# Autodesk Inventor assembly: v1_assem
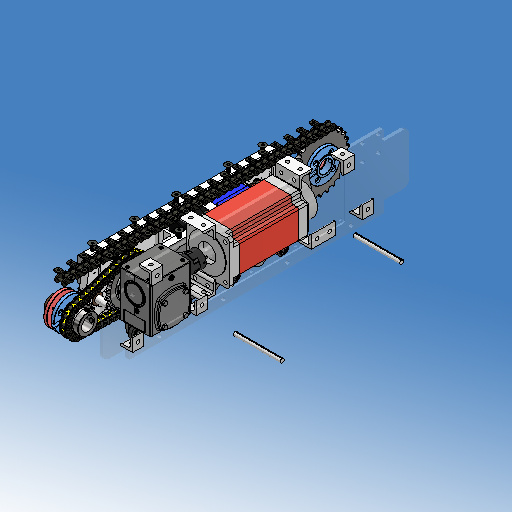
[picture p0: Inventor's stored thumbnail of the model, 512x512]
Saved by Autodesk Inventor 2025 (Build 290162000, 162)
## iProperties
Created: 2022-07-26
Part Number: v1_assem
Document SubType Name: Assembly
Designer: kumpu
Mass: 23927.4 g
Surface Area: 24107.2 cm^2
Volume: 6864.77 cm^3
Author: kumpu
## Documents named in this file (57)
- C:\Users\seene\OneDrive\SBRT\Robocup Rescue\Drive\v1\v1_assem.iam
- C:\Users\seene\OneDrive\SBRT\Robocup Rescue\Drive\v1\Placeholder_ChassisMain.ipt
- C:\Users\seene\OneDrive\SBRT\Robocup Rescue\Drive\v1\5887K172_Right-Angle Speed Reducer.ipt
- C:\Users\seene\OneDrive\SBRT\Robocup Rescue\Drive\v1\QCI-34HC-3_v2.ipt
- C:\Users\seene\OneDrive\SBRT\Robocup Rescue\Drive\v1\Dimensions(Roughly).ipt
- C:\Users\seene\OneDrive\SBRT\Robocup Rescue\Drive\v1\3 Stage HD - CIM Sport.iam
- C:\Users\seene\OneDrive\SBRT\Robocup Rescue\Drive\v1\50XX.ipt
- C:\Users\seene\OneDrive\SBRT\Robocup Rescue\Drive\v1\9939T12_Durometer 64D Spider for 1-5 16 OD Set Screw Vibrate-Damping Precision Flexible Shaft Coupling.ipt
- C:\Users\seene\OneDrive\SBRT\Robocup Rescue\Drive\v1\9939T102_Vibrate-Damping Precision Flexible Shaft Coupling.ipt
- C:\Users\seene\OneDrive\SBRT\Robocup Rescue\Drive\v1\9939T104_Vibrate-Damping Precision Flexible Shaft Coupling.ipt
- C:\Users\seene\OneDrive\SBRT\Robocup Rescue\Drive\v1\Bevels_assem.iam
- C:\Users\seene\OneDrive\SBRT\Robocup Rescue\Drive\v1\ChassisInterface.ipt
- C:\Users\seene\OneDrive\SBRT\Robocup Rescue\Drive\v1\TopPlate.ipt
- C:\Users\seene\OneDrive\SBRT\Robocup Rescue\Drive\v1\6836N166_Flat Sprocket.ipt
- C:\Users\seene\OneDrive\SBRT\Robocup Rescue\Drive\v1\2299K28_Flat Sprocket.ipt
- C:\Users\seene\OneDrive\SBRT\Robocup Rescue\Drive\v1\am-0077a 500 Key Hub REV3.ipt
- C:\Users\seene\OneDrive\SBRT\Robocup Rescue\Drive\v1\6280K675_Roller Chain Sprocket.ipt
- C:\Users\seene\OneDrive\SBRT\Robocup Rescue\Drive\v1\95412A316_18-8 Stainless Steel Threaded Rod.ipt
- C:\Users\seene\OneDrive\SBRT\Robocup Rescue\Drive\v1\91259A585_Alloy Steel Shoulder Screw.ipt
- C:\Users\seene\OneDrive\SBRT\Robocup Rescue\Drive\v1\96505A116_Steel Oversized Washer.ipt
- C:\Users\seene\OneDrive\SBRT\Robocup Rescue\Drive\v1\96282A101_High-Strength Steel Serrated Flange Locknut.ipt
- C:\Users\seene\OneDrive\SBRT\Robocup Rescue\Drive\v1\rubberWasher1.ipt
- C:\Users\seene\OneDrive\SBRT\Robocup Rescue\Drive\v1\trackpath.ipt
- C:\Users\seene\OneDrive\SBRT\Robocup Rescue\Drive\v1\Flipper\chain_male v7.ipt
- C:\Users\seene\OneDrive\SBRT\Robocup Rescue\Drive\v1\Flipper\chain_female v7.ipt
- C:\Users\seene\OneDrive\SBRT\Robocup Rescue\Drive\v1\5055MotorBlock.ipt
- C:\Users\seene\OneDrive\SBRT\Robocup Rescue\Drive\v1\7779T391_Low-Carbon Steel U-Channel.ipt
- C:\Users\seene\OneDrive\SBRT\Robocup Rescue\Drive\v1\am-2460 35 Tooth CIM Gear.ipt
- C:\Users\seene\OneDrive\SBRT\Robocup Rescue\Drive\v1\Flipper\rigid mount shoulder side.ipt
- C:\Users\seene\OneDrive\SBRT\Robocup Rescue\Drive\v1\Flipper\rigid mount threaded side.ipt
- C:\Users\seene\OneDrive\SBRT\Robocup Rescue\Drive\v1\57155K324_Stainless Steel Ball Bearing.ipt
- C:\Users\seene\OneDrive\SBRT\Robocup Rescue\Drive\v1\Spur Gear (28 teeth).ipt
- C:\Users\seene\OneDrive\SBRT\Robocup Rescue\Drive\v1\am-2352 50 Tooth 20 DP 0.75 in. Hex Bore Steel Gear.ipt
- C:\Users\seene\OneDrive\SBRT\Robocup Rescue\Drive\v1\V-Slot wheel.ipt
- C:\Users\seene\OneDrive\SBRT\Robocup Rescue\Drive\v1\91239A241_Button Head Hex Drive Screw.ipt
- C:\Users\seene\OneDrive\SBRT\Robocup Rescue\Drive\v1\6153K15_Stainless Steel Ball Bearing.ipt
- C:\Users\seene\OneDrive\SBRT\Robocup Rescue\Drive\v1\98688A115_General Purpose Zinc-Plated Steel Washer.ipt
- C:\Users\seene\OneDrive\SBRT\Robocup Rescue\Drive\v1\4416T771_Easy-to-Machine 1215 Carbon Steel.ipt
- C:\Users\seene\OneDrive\SBRT\Robocup Rescue\Drive\v1\2868T203_High-Load Oil-Embedded 863 Sleeve Bearing.ipt
- C:\Users\seene\OneDrive\SBRT\Robocup Rescue\Drive\v1\1439K211_1045 Carbon Steel Keyed Rotary Shaft.ipt
- C:\Users\seene\OneDrive\SBRT\Robocup Rescue\Drive\v1\am-0185 45 Tooth Gear 20 dp 500 Hex Bore.ipt
- C:\Users\seene\OneDrive\SBRT\Robocup Rescue\Drive\v1\2938T738_High-Load Oil-Embedded Sleeve Bearing.ipt
- C:\Users\seene\OneDrive\SBRT\Robocup Rescue\Drive\v1\2868T9_High-Load Oil-Embedded 863 Sleeve Bearing.ipt
- C:\Users\seene\OneDrive\SBRT\Robocup Rescue\Drive\v1\2938T12_High-Load Oil-Embedded Sleeve Bearing.ipt
- C:\Users\seene\OneDrive\SBRT\Robocup Rescue\Drive\v1\97175A383_Pull-Out Dowel Pin.ipt
- C:\Users\seene\OneDrive\SBRT\Robocup Rescue\Drive\v1\47065T236_Silver Corner Bracket.ipt
- C:\Users\seene\OneDrive\SBRT\Robocup Rescue\Drive\v1\47065T237_T-Slotted Framing.ipt
- C:\Users\seene\OneDrive\SBRT\Robocup Rescue\Drive\v1\40 chain link.ipt
- C:\Users\seene\OneDrive\SBRT\Robocup Rescue\Drive\v1\ChainPath.ipt
- C:\Users\seene\OneDrive\SBRT\Robocup Rescue\Drive\v1\OuterDriveRail.ipt
- C:\Users\seene\OneDrive\SBRT\Robocup Rescue\Drive\v1\InnerDriveRail.ipt
- C:\Users\seene\OneDrive\SBRT\Robocup Rescue\Drive\v1\TreadGuide.ipt
- C:\Users\seene\OneDrive\SBRT\Robocup Rescue\Drive\v1\TANK flipper\91263A553_Zinc-Plated Alloy Steel Hex Drive Flat Head Screw v1.ipt
- C:\Users\seene\OneDrive\SBRT\Robocup Rescue\Drive\v1\TANK flipper\driveshaftsupport_A.ipt
- C:\Users\seene\OneDrive\SBRT\Robocup Rescue\Drive\v1\TANK flipper\94328A911_Black Oxide Alloy Steel Low-Profile Shoulder Screw v2.ipt
- C:\Users\seene\OneDrive\SBRT\Robocup Rescue\Drive\v1\TankFlipper Flipped.iam
- C:\Users\seene\OneDrive\SBRT\Robocup Rescue\Drive\v1\TankFlipper.iam
## Components (240 placed, 56 different names)
1. Dimensions(Roughly):1 — Flush:9, Flush:10, Flush:11
2. trackpath:1 — Angle:6, Angle:7, Mate:108, Angle:8, Mate:110, Angle:9
3. TankFlipper Flipped:1 [sub-assembly] — Rotational:17
4. TankFlipper:1 [sub-assembly] — Rotational:18
5. Placeholder_ChassisMain:1 — Mate:17, Mate:18, Flush:5, Angle:2, Flush:7, Flush:9, Flush:10, Flush:11, Mate:47, Mate:50, Mate:94, Mate:95, Mate:96, Flush:103, Mate:100, Flush:83, Mate:118, Mate:120
6. 2868T203_High-Load Oil-Embedded 863 Sleeve Bearing:2 — Flush:178, Mate:172, Mate:175, Rotational:12
7. 2868T203_High-Load Oil-Embedded 863 Sleeve Bearing:1 — Flush:178
8. rigid mount threaded side:2 — Mate:140, Mate:141
9. rigid mount shoulder side:2 — Mate:140, Mate:141
10. rigid mount threaded side:1 — Insert:32, Mate:124, Mate:172, Mate:175
11. rigid mount shoulder side:1 — Insert:31, Mate:124, Mate:133, Rotational:17
12. 6280K675_Roller Chain Sprocket:1 — Flush:99, Flush:180, Mate:173, Rotational:18
13. 2299K28_Flat Sprocket:1 — Mate:87, Insert:21, Flush:99
14. am-0077a 500 Key Hub REV3:1 — Mate:87, Insert:21, Flush:100, Mate:88
15. 6836N166_Flat Sprocket:2 — Angle:4, Insert:31, Insert:32
16. 9939T12_Durometer 64D Spider for 1-5 16 OD Set Screw Vibrate-Damping Precision Flexible Shaft Coupling:2
17. 9939T102_Vibrate-Damping Precision Flexible Shaft Coupling:2 — Mate:31, Flush:110
18. 9939T104_Vibrate-Damping Precision Flexible Shaft Coupling:2
19. QCI-34HC-3_v2:2 — Mate:20, Flush:109, Mate:165, Angle:39, Mate:187
20. 5887K172_Right-Angle Speed Reducer:1 — Angle:2, Flush:7, Mate:20, Flush:110, Mate:31, Mate:47, Flush:100, Mate:88, Mate:139, Flush:163
21. 47065T236_Silver Corner Bracket:8 — Mate:200, Flush:211, Flush:212
22. 47065T236_Silver Corner Bracket:3 — Mate:179, Mate:182, Flush:197, Flush:198
23. 47065T236_Silver Corner Bracket:4 — Mate:180, Flush:182, Mate:184, Flush:186, Flush:189
24. 47065T236_Silver Corner Bracket:5 — Mate:181, Flush:182, Mate:185
25. 47065T237_T-Slotted Framing:5 — Flush:186, Flush:187, Flush:188, Flush:202, Flush:203, Flush:209
26. 47065T236_Silver Corner Bracket:6 — Mate:186, Flush:188, Flush:189
27. 47065T236_Silver Corner Bracket:7 — Mate:187, Mate:188, Flush:205, Flush:210
28. 47065T237_T-Slotted Framing:6 — Mate:189, Flush:198, Mate:190, Flush:209, Flush:210, Flush:211, Flush:212
29. 47065T237_T-Slotted Framing:8 — Flush:202, Flush:203, Mate:191, Flush:204
30. 47065T237_T-Slotted Framing:9 — Mate:192, Flush:204, Flush:205, Mate:193
31. 47065T236_Silver Corner Bracket:2 — Flush:174, Flush:175, Flush:176
32. 47065T236_Silver Corner Bracket:1 — Flush:174, Flush:175, Flush:177, Mate:169, Mate:170
33. 57155K324_Stainless Steel Ball Bearing:3 — Flush:141
34. 57155K324_Stainless Steel Ball Bearing:4 — Flush:140, Mate:152, Insert:49
35. 57155K324_Stainless Steel Ball Bearing:2 — Mate:126, Flush:130, Mate:150, Flush:140, Mate:156, Insert:50
36. 57155K324_Stainless Steel Ball Bearing:1 — Mate:126, Mate:127, Flush:129, Flush:141
37. 47065T237_T-Slotted Framing:2 — Flush:167, Mate:165, Mate:166, Flush:170
38. 47065T237_T-Slotted Framing:3 — Flush:170, Mate:167, Flush:172, Flush:173
39. 47065T237_T-Slotted Framing:1 — Flush:168, Flush:171
40. 47065T237_T-Slotted Framing:4 — Flush:171, Flush:172, Flush:187
41. 7779T391_Low-Carbon Steel U-Channel:1 — Mate:119, Mate:120, Flush:129, Flush:130, Insert:38, Insert:43, Flush:142, Angle:38, Flush:166, Flush:167, Flush:168, Mate:166, Mate:167, Flush:173, Mate:186, Flush:206, Mate:194, Mate:195, Insert:51, Insert:52, Mate:196
42. TopPlate:2 — Flush:83, Flush:107, Flush:138, Flush:139, Mate:170, Mate:191, Mate:192, Mate:197
43. ChassisInterface:2 — Mate:50, Flush:107, Angle:5, Flush:138, Flush:139, Mate:139, Mate:149, Mate:150, Flush:163, Flush:176, Flush:177, Mate:169, Angle:39, Mate:179, Mate:180, Mate:181, Mate:188, Flush:197, Mate:189, Mate:193, Mate:197, Angle:41
44. 4416T771_Easy-to-Machine 1215 Carbon Steel:1 — Insert:44, Insert:45, Angle:35, Mate:157
45. 2938T12_High-Load Oil-Embedded Sleeve Bearing:1 — Insert:45
46. Bevels_assem:3 [sub-assembly] — Mate:38, Angle:31, Mate:127, Mate:128
47. 5055MotorBlock:1 — Insert:27, Mate:115, Insert:28, Angle:10
48. am-2460 35 Tooth CIM Gear:2 — Mate:128, Flush:131, Mate:131, Flush:134
49. 1439K211_1045 Carbon Steel Keyed Rotary Shaft:2 — Insert:50
50. am-0185 45 Tooth Gear 20 dp 500 Hex Bore:1 — Mate:155, Mate:156, Flush:142, Insert:48
51. 97175A383_Pull-Out Dowel Pin:2 — Flush:164, Flush:165, Mate:162, Flush:166
52. 2868T9_High-Load Oil-Embedded 863 Sleeve Bearing:1 — Insert:48, Mate:162
53. 97175A383_Pull-Out Dowel Pin:1 — Flush:165, Mate:163
54. 2938T738_High-Load Oil-Embedded Sleeve Bearing:1 — Insert:44, Mate:158, Mate:163
55. Spur Gear (28 teeth):1 — Mate:131, Flush:133, Mate:134, Mate:135, Angle:33, Angle:35, Mate:158, Angle:38, Flush:162
56. am-2352 50 Tooth 20 DP 0.75 in. Hex Bore Steel Gear:1 — Flush:134, Mate:134, Mate:135, Angle:33, Flush:137, Mate:155, Mate:157
57. 50XX:3 — Insert:27, Mate:115
58. 3 Stage HD - CIM Sport:3 [sub-assembly] — Mate:33, Mate:38, Angle:5, Insert:28, Angle:10, Flush:111
59. 5055MotorBlock:2 — Insert:29, Mate:116, Mate:117, Insert:30
60. 2938T12_High-Load Oil-Embedded Sleeve Bearing:2 — Mate:160
61. 4416T771_Easy-to-Machine 1215 Carbon Steel:2 — Angle:36, Mate:159
62. 50XX:4 — Insert:29, Mate:116, Mate:118
63. 3 Stage HD - CIM Sport:4 [sub-assembly] — Mate:33, Mate:39, Mate:117, Insert:30, Flush:109, Angle:11, Flush:111
64. Bevels_assem:4 [sub-assembly] — Mate:39, Angle:31, Angle:11, Mate:121, Angle:32
65. am-2460 35 Tooth CIM Gear:1 — Mate:121, Angle:32, Flush:131, Mate:132, Mate:152
66. 1439K211_1045 Carbon Steel Keyed Rotary Shaft:1 — Insert:49, Mate:149
67. Spur Gear (28 teeth):2 — Flush:133, Mate:132, Mate:133, Mate:137, Angle:36, Angle:37, Flush:162
68. 2938T738_High-Load Oil-Embedded Sleeve Bearing:2 — Mate:161
69. 97175A383_Pull-Out Dowel Pin:3 — Mate:161, Flush:164
70. am-2352 50 Tooth 20 DP 0.75 in. Hex Bore Steel Gear:2 — Mate:137, Flush:137, Angle:37, Mate:159, Mate:160
71. driveshaftsupport_A:2 — Rotational:13
72. driveshaftsupport_A:1 — Flush:213, Flush:214, Rotational:12
73. 94328A911_Black Oxide Alloy Steel Low-Profile Shoulder Screw v2:1 — Rotational:11
74. 94328A911_Black Oxide Alloy Steel Low-Profile Shoulder Screw v2:2 — Rotational:10
75. 94328A911_Black Oxide Alloy Steel Low-Profile Shoulder Screw v2:3 — Insert:53, Rotational:15
76. 94328A911_Black Oxide Alloy Steel Low-Profile Shoulder Screw v2:4 — Rotational:14
77. OuterDriveRail:1 — Flush:206, Mate:194, Mate:196, Flush:208, Mate:198, Mate:199, Flush:213, Flush:214, Rotational:10, Rotational:11, Rotational:13, Rotational:14, Insert:53, Rotational:15
78. InnerDriveRail:1 — Mate:195, Insert:51, Insert:52, Mate:200
79. 91263A553_Zinc-Plated Alloy Steel Hex Drive Flat Head Screw v1:6 — Rotational:6
80. 91263A553_Zinc-Plated Alloy Steel Hex Drive Flat Head Screw v1:7 — Rotational:7
81. 91263A553_Zinc-Plated Alloy Steel Hex Drive Flat Head Screw v1:8 — Rotational:8
82. 91263A553_Zinc-Plated Alloy Steel Hex Drive Flat Head Screw v1:9 — Rotational:9
83. 91263A553_Zinc-Plated Alloy Steel Hex Drive Flat Head Screw v1:1 — Rotational:5
84. 91263A553_Zinc-Plated Alloy Steel Hex Drive Flat Head Screw v1:2 — Rotational:1
85. 91263A553_Zinc-Plated Alloy Steel Hex Drive Flat Head Screw v1:3 — Rotational:2
86. 91263A553_Zinc-Plated Alloy Steel Hex Drive Flat Head Screw v1:4 — Rotational:3
87. 91263A553_Zinc-Plated Alloy Steel Hex Drive Flat Head Screw v1:5 — Rotational:4
88. TreadGuide:1 — Flush:208, Mate:198, Mate:199, Rotational:1, Rotational:2, Rotational:3, Rotational:4, Rotational:5, Rotational:6, Rotational:7, Rotational:8, Rotational:9
89. ChainPath:1 — Flush:180, Mate:174, Angle:40
90. 95412A316_18-8 Stainless Steel Threaded Rod:1 — Mate:96, Flush:103, Mate:99
91. 91259A585_Alloy Steel Shoulder Screw:1 — Mate:94, Mate:95, Insert:23
92. 96505A116_Steel Oversized Washer:1 — Insert:23, Insert:24
93. 96282A101_High-Strength Steel Serrated Flange Locknut:1 — Mate:99, Mate:100, Mate:182, Mate:190
94. rubberWasher1:1 — Insert:24
95. 91259A585_Alloy Steel Shoulder Screw:2 — Insert:25
96. 96505A116_Steel Oversized Washer:2 — Insert:25, Insert:26
97. 96282A101_High-Strength Steel Serrated Flange Locknut:2
98. rubberWasher1:2 — Insert:26
99. 95412A316_18-8 Stainless Steel Threaded Rod:2
100. 91259A585_Alloy Steel Shoulder Screw:3
101. 96505A116_Steel Oversized Washer:3
102. 96282A101_High-Strength Steel Serrated Flange Locknut:3
103. rubberWasher1:3
104. 91259A585_Alloy Steel Shoulder Screw:4
105. 96505A116_Steel Oversized Washer:4
106. 96282A101_High-Strength Steel Serrated Flange Locknut:4
107. rubberWasher1:4
108. 95412A316_18-8 Stainless Steel Threaded Rod:3
109. 91259A585_Alloy Steel Shoulder Screw:5
110. 96505A116_Steel Oversized Washer:5
111. 96282A101_High-Strength Steel Serrated Flange Locknut:5 — Mate:184
112. rubberWasher1:5
113. 91259A585_Alloy Steel Shoulder Screw:6
114. 96505A116_Steel Oversized Washer:6
115. 96282A101_High-Strength Steel Serrated Flange Locknut:6
116. rubberWasher1:6
117. 95412A316_18-8 Stainless Steel Threaded Rod:4
118. 91259A585_Alloy Steel Shoulder Screw:7
119. 96505A116_Steel Oversized Washer:7
120. 96282A101_High-Strength Steel Serrated Flange Locknut:7 — Mate:185
121. rubberWasher1:7
122. 91259A585_Alloy Steel Shoulder Screw:8
123. 96505A116_Steel Oversized Washer:8
124. 96282A101_High-Strength Steel Serrated Flange Locknut:8
125. rubberWasher1:8
126. 91239A241_Button Head Hex Drive Screw:2
127. V-Slot wheel:2
128. 6153K15_Stainless Steel Ball Bearing:3
129. 98688A115_General Purpose Zinc-Plated Steel Washer:2 — Insert:43
130. 6153K15_Stainless Steel Ball Bearing:4
131. V-Slot wheel:1 — Insert:34, Insert:35, Tangent:1
132. 91239A241_Button Head Hex Drive Screw:1 — Insert:36
133. 6153K15_Stainless Steel Ball Bearing:1 — Insert:35, Insert:36
134. 98688A115_General Purpose Zinc-Plated Steel Washer:1 — Insert:37, Insert:38
135. 6153K15_Stainless Steel Ball Bearing:2 — Insert:34, Insert:37
136. 91239A241_Button Head Hex Drive Screw:3
137. V-Slot wheel:3
138. 6153K15_Stainless Steel Ball Bearing:5
139. 98688A115_General Purpose Zinc-Plated Steel Washer:3
140. 6153K15_Stainless Steel Ball Bearing:6
141. V-Slot wheel:4
142. 91239A241_Button Head Hex Drive Screw:4
143. 6153K15_Stainless Steel Ball Bearing:7
144. 98688A115_General Purpose Zinc-Plated Steel Washer:4
145. 6153K15_Stainless Steel Ball Bearing:8
146. 91239A241_Button Head Hex Drive Screw:5
147. V-Slot wheel:5
148. 6153K15_Stainless Steel Ball Bearing:9
149. 98688A115_General Purpose Zinc-Plated Steel Washer:5
150. 6153K15_Stainless Steel Ball Bearing:10
151. V-Slot wheel:6
152. 91239A241_Button Head Hex Drive Screw:6
153. 6153K15_Stainless Steel Ball Bearing:11
154. 98688A115_General Purpose Zinc-Plated Steel Washer:6
155. 6153K15_Stainless Steel Ball Bearing:12
156. 91239A241_Button Head Hex Drive Screw:7
157. V-Slot wheel:7
158. 6153K15_Stainless Steel Ball Bearing:13
159. 98688A115_General Purpose Zinc-Plated Steel Washer:7
160. 6153K15_Stainless Steel Ball Bearing:14
161. V-Slot wheel:8
162. 91239A241_Button Head Hex Drive Screw:8
163. 6153K15_Stainless Steel Ball Bearing:15
164. 98688A115_General Purpose Zinc-Plated Steel Washer:8
165. 6153K15_Stainless Steel Ball Bearing:16
166. chain_male v7:1 — Mate:110, Mate:111, Angle:9
167. chain_female v7:1 — Mate:108, Angle:8, Mate:111
168. chain_male v7:2
169. chain_female v7:4
170. chain_male v7:3
171. chain_female v7:5
172. chain_male v7:4
173. chain_female v7:6
174. chain_male v7:5
175. chain_female v7:7
176. chain_male v7:6
177. chain_female v7:8
178. chain_male v7:7
179. chain_female v7:9
180. chain_male v7:8
181. chain_female v7:10
182. chain_male v7:9
183. chain_female v7:11
184. chain_male v7:10
185. chain_female v7:12
186. chain_male v7:11
187. chain_female v7:13
188. chain_male v7:12
189. chain_female v7:14
190. chain_male v7:13
191. chain_female v7:15
192. chain_male v7:14
193. chain_female v7:16
194. chain_male v7:15
195. chain_female v7:17
196. chain_male v7:16
197. chain_female v7:18
198. chain_male v7:17
199. chain_female v7:19
200. chain_male v7:18
201. chain_female v7:20
202. chain_male v7:19
203. chain_female v7:21
204. chain_male v7:20
205. chain_female v7:22
206. chain_male v7:21
207. chain_female v7:23
208. 40 chain link:1 — Mate:173, Mate:174, Angle:40
209. 40 chain link:2
210. 40 chain link:3
211. 40 chain link:4
212. 40 chain link:5
213. 40 chain link:6
214. 40 chain link:7
215. 40 chain link:8
216. 40 chain link:9
217. 40 chain link:10
218. 40 chain link:11
219. 40 chain link:12
220. 40 chain link:13
221. 40 chain link:14
222. 40 chain link:15
223. 40 chain link:16
224. 40 chain link:17
225. 40 chain link:18
226. 40 chain link:19
227. 40 chain link:20
228. 40 chain link:21
229. 40 chain link:22
230. 40 chain link:23
231. 40 chain link:24
232. 40 chain link:25
233. 40 chain link:26
234. 40 chain link:27
235. 40 chain link:28
236. 40 chain link:29
237. 40 chain link:30
238. 40 chain link:31
239. 40 chain link:32
240. 40 chain link:33
## Component patterns: (4 elements, first: 95412A316_18-8 Stainless Steel Threaded Rod:1 + 91259A585_Alloy Steel Shoulder Screw:1 + 96505A116_Steel Oversized Washer:1 + 96282A101_High-Strength Steel Serrated Flange Locknut:1 + rubberWasher1:1 + 91259A585_Alloy Steel Shoulder Screw:2 + 96505A116_Steel Oversized Washer:2 + 96282A101_High-Strength Steel Serrated Flange Locknut:2 + rubberWasher1:2), (4 elements, first: 91239A241_Button Head Hex Drive Screw:2 + V-Slot wheel:2 + 6153K15_Stainless Steel Ball Bearing:3 + 98688A115_General Purpose Zinc-Plated Steel Washer:2 + 6153K15_Stainless Steel Ball Bearing:4 + V-Slot wheel:1 + 91239A241_Button Head Hex Drive Screw:1 + 6153K15_Stainless Steel Ball Bearing:1 + 98688A115_General Purpose Zinc-Plated Steel Washer:1 + 6153K15_Stainless Steel Ball Bearing:2), (21 elements, first: chain_male v7:1 + chain_female v7:1), (33 elements, first: 40 chain link:1)
## Relationships (215: Mate 84, Flush 61, Insert 33, Angle 19, RevoluteJoint 17, Tangent 1)
- Flush:2 (-31.75 mm)
- Mate:17: Placeholder_ChassisMain:1
- Mate:18: Placeholder_ChassisMain:1
- Flush:5: Placeholder_ChassisMain:1
- Angle:2 (0 deg): Placeholder_ChassisMain:1 ↔ 5887K172_Right-Angle Speed Reducer:1
- Flush:7 (3.175 mm): Placeholder_ChassisMain:1 ↔ 5887K172_Right-Angle Speed Reducer:1
- Mate:20: QCI-34HC-3_v2:2 ↔ 5887K172_Right-Angle Speed Reducer:1
- Flush:9: Dimensions(Roughly):1 ↔ Placeholder_ChassisMain:1
- Flush:10: Dimensions(Roughly):1 ↔ Placeholder_ChassisMain:1
- Flush:11 (-63.5 mm): Dimensions(Roughly):1 ↔ Placeholder_ChassisMain:1
- Flush:110 (9.525 mm): 9939T102_Vibrate-Damping Precision Flexible Shaft Coupling:2 ↔ 5887K172_Right-Angle Speed Reducer:1
- [Insert]: 9939T12_Durometer 64D Spider for 1-5 16 OD Set Screw Vibrate-Damping Precision Flexible Shaft Coupling:2 ↔ 9939T102_Vibrate-Damping Precision Flexible Shaft Coupling:2
- [Insert]: 9939T12_Durometer 64D Spider for 1-5 16 OD Set Screw Vibrate-Damping Precision Flexible Shaft Coupling:2 ↔ 9939T104_Vibrate-Damping Precision Flexible Shaft Coupling:2
- [Mate] (0.6858 mm): 9939T12_Durometer 64D Spider for 1-5 16 OD Set Screw Vibrate-Damping Precision Flexible Shaft Coupling:2 ↔ 9939T102_Vibrate-Damping Precision Flexible Shaft Coupling:2
- [Mate] (0.6858 mm): 9939T12_Durometer 64D Spider for 1-5 16 OD Set Screw Vibrate-Damping Precision Flexible Shaft Coupling:2 ↔ 9939T104_Vibrate-Damping Precision Flexible Shaft Coupling:2
- Mate:31: 9939T102_Vibrate-Damping Precision Flexible Shaft Coupling:2 ↔ 5887K172_Right-Angle Speed Reducer:1
- Mate:33 (3.175 mm): 3 Stage HD - CIM Sport:3 ↔ 3 Stage HD - CIM Sport:4
- Mate:38: Bevels_assem:3 ↔ 3 Stage HD - CIM Sport:3
- Mate:39: 3 Stage HD - CIM Sport:4 ↔ Bevels_assem:4
- Angle:31 (0 deg): Bevels_assem:3 ↔ Bevels_assem:4
- Mate:47 (24.13 mm): Placeholder_ChassisMain:1 ↔ 5887K172_Right-Angle Speed Reducer:1
- Mate:50: Placeholder_ChassisMain:1 ↔ ChassisInterface:2
- Flush:83: Placeholder_ChassisMain:1 ↔ TopPlate:2
- Flush:107: TopPlate:2 ↔ ChassisInterface:2
- Mate:87: 2299K28_Flat Sprocket:1 ↔ am-0077a 500 Key Hub REV3:1
- Insert:21: 2299K28_Flat Sprocket:1 ↔ am-0077a 500 Key Hub REV3:1
- Flush:99: 6280K675_Roller Chain Sprocket:1 ↔ 2299K28_Flat Sprocket:1
- Flush:100 (3.175 mm): am-0077a 500 Key Hub REV3:1 ↔ 5887K172_Right-Angle Speed Reducer:1
- Mate:88: am-0077a 500 Key Hub REV3:1 ↔ 5887K172_Right-Angle Speed Reducer:1
- Mate:94: Placeholder_ChassisMain:1 ↔ 91259A585_Alloy Steel Shoulder Screw:1
- Mate:95: Placeholder_ChassisMain:1 ↔ 91259A585_Alloy Steel Shoulder Screw:1
- Mate:96: Placeholder_ChassisMain:1 ↔ 95412A316_18-8 Stainless Steel Threaded Rod:1
- Flush:103 (-12.7 mm): Placeholder_ChassisMain:1 ↔ 95412A316_18-8 Stainless Steel Threaded Rod:1
- Insert:23: 91259A585_Alloy Steel Shoulder Screw:1 ↔ 96505A116_Steel Oversized Washer:1
- Mate:99: 95412A316_18-8 Stainless Steel Threaded Rod:1 ↔ 96282A101_High-Strength Steel Serrated Flange Locknut:1
- Mate:100 (6.35 mm): Placeholder_ChassisMain:1 ↔ 96282A101_High-Strength Steel Serrated Flange Locknut:1
- Insert:24: 96505A116_Steel Oversized Washer:1 ↔ rubberWasher1:1
- Insert:25: 91259A585_Alloy Steel Shoulder Screw:2 ↔ 96505A116_Steel Oversized Washer:2
- Insert:26: 96505A116_Steel Oversized Washer:2 ↔ rubberWasher1:2
- Angle:4 (20 deg): 6836N166_Flat Sprocket:2
- Angle:5 (0 deg): ChassisInterface:2 ↔ 3 Stage HD - CIM Sport:3
- Angle:6 (0 deg): trackpath:1
- Angle:7 (0 deg): trackpath:1
- Mate:108: trackpath:1 ↔ chain_female v7:1
- Angle:8 (90 deg): trackpath:1 ↔ chain_female v7:1
- Mate:110: trackpath:1 ↔ chain_male v7:1
- Mate:111: chain_male v7:1 ↔ chain_female v7:1
- Angle:9 (-90 deg): trackpath:1 ↔ chain_male v7:1
- Insert:27: 5055MotorBlock:1 ↔ 50XX:3
- Mate:115: 5055MotorBlock:1 ↔ 50XX:3
- Insert:28: 5055MotorBlock:1 ↔ 3 Stage HD - CIM Sport:3
- Angle:10 (0 deg): 5055MotorBlock:1 ↔ 3 Stage HD - CIM Sport:3
- Insert:29: 5055MotorBlock:2 ↔ 50XX:4
- Mate:116: 5055MotorBlock:2 ↔ 50XX:4
- Mate:117: 5055MotorBlock:2 ↔ 3 Stage HD - CIM Sport:4
- Insert:30: 5055MotorBlock:2 ↔ 3 Stage HD - CIM Sport:4
- Flush:109: QCI-34HC-3_v2:2 ↔ 3 Stage HD - CIM Sport:4
- Angle:11 (0 deg): 3 Stage HD - CIM Sport:4 ↔ Bevels_assem:4
- Mate:118 (127 mm): Placeholder_ChassisMain:1 ↔ 50XX:4
- Mate:119 (-152.4 mm): 7779T391_Low-Carbon Steel U-Channel:1
- Mate:120 (101.6 mm): Placeholder_ChassisMain:1 ↔ 7779T391_Low-Carbon Steel U-Channel:1
- Mate:121: Bevels_assem:4 ↔ am-2460 35 Tooth CIM Gear:1
- Angle:32 (0 deg): Bevels_assem:4 ↔ am-2460 35 Tooth CIM Gear:1
- Flush:111: 3 Stage HD - CIM Sport:3 ↔ 3 Stage HD - CIM Sport:4
- Insert:31: rigid mount shoulder side:1 ↔ 6836N166_Flat Sprocket:2
- Insert:32: rigid mount threaded side:1 ↔ 6836N166_Flat Sprocket:2
- Mate:124: rigid mount threaded side:1 ↔ rigid mount shoulder side:1
- Mate:126: 57155K324_Stainless Steel Ball Bearing:2 ↔ 57155K324_Stainless Steel Ball Bearing:1
- Mate:127: 57155K324_Stainless Steel Ball Bearing:1 ↔ Bevels_assem:3
- Flush:129: 57155K324_Stainless Steel Ball Bearing:1 ↔ 7779T391_Low-Carbon Steel U-Channel:1
- Flush:130: 57155K324_Stainless Steel Ball Bearing:2 ↔ 7779T391_Low-Carbon Steel U-Channel:1
- Mate:128: Bevels_assem:3 ↔ am-2460 35 Tooth CIM Gear:2
- Flush:131: am-2460 35 Tooth CIM Gear:2 ↔ am-2460 35 Tooth CIM Gear:1
- Mate:131 (53.975 mm): am-2460 35 Tooth CIM Gear:2 ↔ Spur Gear (28 teeth):1
- Flush:133: Spur Gear (28 teeth):1 ↔ Spur Gear (28 teeth):2
- Mate:132 (53.975 mm): am-2460 35 Tooth CIM Gear:1 ↔ Spur Gear (28 teeth):2
- Mate:133 (79.375 mm): rigid mount shoulder side:1 ↔ Spur Gear (28 teeth):2
- Flush:134: am-2460 35 Tooth CIM Gear:2 ↔ am-2352 50 Tooth 20 DP 0.75 in. Hex Bore Steel Gear:1
- Mate:134: Spur Gear (28 teeth):1 ↔ am-2352 50 Tooth 20 DP 0.75 in. Hex Bore Steel Gear:1
- Mate:135 (2.54 mm): Spur Gear (28 teeth):1 ↔ am-2352 50 Tooth 20 DP 0.75 in. Hex Bore Steel Gear:1
- Angle:33 (0 deg): Spur Gear (28 teeth):1 ↔ am-2352 50 Tooth 20 DP 0.75 in. Hex Bore Steel Gear:1
- Mate:137: Spur Gear (28 teeth):2 ↔ am-2352 50 Tooth 20 DP 0.75 in. Hex Bore Steel Gear:2
- Flush:137: am-2352 50 Tooth 20 DP 0.75 in. Hex Bore Steel Gear:1 ↔ am-2352 50 Tooth 20 DP 0.75 in. Hex Bore Steel Gear:2
- Insert:34: V-Slot wheel:1 ↔ 6153K15_Stainless Steel Ball Bearing:2
- Insert:35: V-Slot wheel:1 ↔ 6153K15_Stainless Steel Ball Bearing:1
- Insert:36: 91239A241_Button Head Hex Drive Screw:1 ↔ 6153K15_Stainless Steel Ball Bearing:1
- Insert:37: 98688A115_General Purpose Zinc-Plated Steel Washer:1 ↔ 6153K15_Stainless Steel Ball Bearing:2
- Insert:38: 7779T391_Low-Carbon Steel U-Channel:1 ↔ 98688A115_General Purpose Zinc-Plated Steel Washer:1
- [Insert]: V-Slot wheel:2 ↔ 6153K15_Stainless Steel Ball Bearing:4
- [Insert]: V-Slot wheel:2 ↔ 6153K15_Stainless Steel Ball Bearing:3
- [Insert]: 91239A241_Button Head Hex Drive Screw:2 ↔ 6153K15_Stainless Steel Ball Bearing:3
- [Insert]: 98688A115_General Purpose Zinc-Plated Steel Washer:2 ↔ 6153K15_Stainless Steel Ball Bearing:4
- Insert:43: 7779T391_Low-Carbon Steel U-Channel:1 ↔ 98688A115_General Purpose Zinc-Plated Steel Washer:2
- Flush:138 (50.8 mm): TopPlate:2 ↔ ChassisInterface:2
- Flush:139 (-25.4 mm): TopPlate:2 ↔ ChassisInterface:2
- Mate:139 (-65.0875 mm): 5887K172_Right-Angle Speed Reducer:1 ↔ ChassisInterface:2
- Mate:140: rigid mount threaded side:2 ↔ rigid mount shoulder side:2
- Mate:141: rigid mount threaded side:2 ↔ rigid mount shoulder side:2
- Mate:149 (-133.35 mm): ChassisInterface:2 ↔ 1439K211_1045 Carbon Steel Keyed Rotary Shaft:1
- Mate:150 (-187.325 mm): 57155K324_Stainless Steel Ball Bearing:2 ↔ ChassisInterface:2
- [Mate]: 57155K324_Stainless Steel Ball Bearing:3 ↔ 57155K324_Stainless Steel Ball Bearing:4
- Flush:140: 57155K324_Stainless Steel Ball Bearing:4 ↔ 57155K324_Stainless Steel Ball Bearing:2
- Flush:141: 57155K324_Stainless Steel Ball Bearing:3 ↔ 57155K324_Stainless Steel Ball Bearing:1
- Mate:152: 57155K324_Stainless Steel Ball Bearing:4 ↔ am-2460 35 Tooth CIM Gear:1
- Mate:155 (60.325 mm): am-0185 45 Tooth Gear 20 dp 500 Hex Bore:1 ↔ am-2352 50 Tooth 20 DP 0.75 in. Hex Bore Steel Gear:1
- Mate:156 (50.8 mm): 57155K324_Stainless Steel Ball Bearing:2 ↔ am-0185 45 Tooth Gear 20 dp 500 Hex Bore:1
- Flush:142 (1.5875 mm): 7779T391_Low-Carbon Steel U-Channel:1 ↔ am-0185 45 Tooth Gear 20 dp 500 Hex Bore:1
- Insert:44: 4416T771_Easy-to-Machine 1215 Carbon Steel:1 ↔ 2938T738_High-Load Oil-Embedded Sleeve Bearing:1
- Insert:45: 4416T771_Easy-to-Machine 1215 Carbon Steel:1 ↔ 2938T12_High-Load Oil-Embedded Sleeve Bearing:1
- Angle:35 (0 deg): 4416T771_Easy-to-Machine 1215 Carbon Steel:1 ↔ Spur Gear (28 teeth):1
- Mate:157: 4416T771_Easy-to-Machine 1215 Carbon Steel:1 ↔ am-2352 50 Tooth 20 DP 0.75 in. Hex Bore Steel Gear:1
- Mate:158: 2938T738_High-Load Oil-Embedded Sleeve Bearing:1 ↔ Spur Gear (28 teeth):1
- [Insert]: 4416T771_Easy-to-Machine 1215 Carbon Steel:2 ↔ 2938T738_High-Load Oil-Embedded Sleeve Bearing:2
- [Insert]: 2938T12_High-Load Oil-Embedded Sleeve Bearing:2 ↔ 4416T771_Easy-to-Machine 1215 Carbon Steel:2
- Angle:36 (0 deg): 4416T771_Easy-to-Machine 1215 Carbon Steel:2 ↔ Spur Gear (28 teeth):2
- Angle:37 (0 deg): Spur Gear (28 teeth):2 ↔ am-2352 50 Tooth 20 DP 0.75 in. Hex Bore Steel Gear:2
- Mate:159: 4416T771_Easy-to-Machine 1215 Carbon Steel:2 ↔ am-2352 50 Tooth 20 DP 0.75 in. Hex Bore Steel Gear:2
- Mate:160: 2938T12_High-Load Oil-Embedded Sleeve Bearing:2 ↔ am-2352 50 Tooth 20 DP 0.75 in. Hex Bore Steel Gear:2
- Insert:48: am-0185 45 Tooth Gear 20 dp 500 Hex Bore:1 ↔ 2868T9_High-Load Oil-Embedded 863 Sleeve Bearing:1
- Angle:38 (0 deg): 7779T391_Low-Carbon Steel U-Channel:1 ↔ Spur Gear (28 teeth):1
- Flush:162: Spur Gear (28 teeth):1 ↔ Spur Gear (28 teeth):2
- Insert:49: 57155K324_Stainless Steel Ball Bearing:4 ↔ 1439K211_1045 Carbon Steel Keyed Rotary Shaft:1
- Insert:50: 57155K324_Stainless Steel Ball Bearing:2 ↔ 1439K211_1045 Carbon Steel Keyed Rotary Shaft:2
- Flush:163 (6.35 mm): 5887K172_Right-Angle Speed Reducer:1 ↔ ChassisInterface:2
- Mate:161: 2938T738_High-Load Oil-Embedded Sleeve Bearing:2 ↔ 97175A383_Pull-Out Dowel Pin:3
- Flush:164: 97175A383_Pull-Out Dowel Pin:2 ↔ 97175A383_Pull-Out Dowel Pin:3
- Flush:165: 97175A383_Pull-Out Dowel Pin:2 ↔ 97175A383_Pull-Out Dowel Pin:1
- Mate:162: 97175A383_Pull-Out Dowel Pin:2 ↔ 2868T9_High-Load Oil-Embedded 863 Sleeve Bearing:1
- Mate:163: 97175A383_Pull-Out Dowel Pin:1 ↔ 2938T738_High-Load Oil-Embedded Sleeve Bearing:1
- Flush:166 (12.7 mm): 7779T391_Low-Carbon Steel U-Channel:1 ↔ 97175A383_Pull-Out Dowel Pin:2
- Flush:167: 47065T237_T-Slotted Framing:2 ↔ 7779T391_Low-Carbon Steel U-Channel:1
- Flush:168: 47065T237_T-Slotted Framing:1 ↔ 7779T391_Low-Carbon Steel U-Channel:1
- Mate:165 (6.35 mm): QCI-34HC-3_v2:2 ↔ 47065T237_T-Slotted Framing:2
- Mate:166: 47065T237_T-Slotted Framing:2 ↔ 7779T391_Low-Carbon Steel U-Channel:1
- Flush:170: 47065T237_T-Slotted Framing:2 ↔ 47065T237_T-Slotted Framing:3
- Mate:167: 47065T237_T-Slotted Framing:3 ↔ 7779T391_Low-Carbon Steel U-Channel:1
- Flush:171: 47065T237_T-Slotted Framing:1 ↔ 47065T237_T-Slotted Framing:4
- Flush:172: 47065T237_T-Slotted Framing:3 ↔ 47065T237_T-Slotted Framing:4
- Flush:173: 47065T237_T-Slotted Framing:3 ↔ 7779T391_Low-Carbon Steel U-Channel:1
- Flush:174: 47065T236_Silver Corner Bracket:2 ↔ 47065T236_Silver Corner Bracket:1
- Flush:175: 47065T236_Silver Corner Bracket:2 ↔ 47065T236_Silver Corner Bracket:1
- Flush:176: 47065T236_Silver Corner Bracket:2 ↔ ChassisInterface:2
- Flush:177: 47065T236_Silver Corner Bracket:1 ↔ ChassisInterface:2
- Mate:169: 47065T236_Silver Corner Bracket:1 ↔ ChassisInterface:2
- Mate:170: 47065T236_Silver Corner Bracket:1 ↔ TopPlate:2
- Flush:178: 2868T203_High-Load Oil-Embedded 863 Sleeve Bearing:2 ↔ 2868T203_High-Load Oil-Embedded 863 Sleeve Bearing:1
- Mate:172: 2868T203_High-Load Oil-Embedded 863 Sleeve Bearing:2 ↔ rigid mount threaded side:1
- Angle:39 (0 deg): QCI-34HC-3_v2:2 ↔ ChassisInterface:2
- Flush:180: 6280K675_Roller Chain Sprocket:1 ↔ ChainPath:1
- Mate:173 (-3.6068 mm): 6280K675_Roller Chain Sprocket:1 ↔ 40 chain link:1
- Mate:174: ChainPath:1 ↔ 40 chain link:1
- Angle:40 (90 deg): ChainPath:1 ↔ 40 chain link:1
- Mate:175 (0.7937 mm): 2868T203_High-Load Oil-Embedded 863 Sleeve Bearing:2 ↔ rigid mount threaded side:1
- Mate:179: 47065T236_Silver Corner Bracket:3 ↔ ChassisInterface:2
- Mate:180: 47065T236_Silver Corner Bracket:4 ↔ ChassisInterface:2
- Mate:181: 47065T236_Silver Corner Bracket:5 ↔ ChassisInterface:2
- Flush:182: 47065T236_Silver Corner Bracket:4 ↔ 47065T236_Silver Corner Bracket:5
- Mate:182 (26.9875 mm): 47065T236_Silver Corner Bracket:3 ↔ 96282A101_High-Strength Steel Serrated Flange Locknut:1
- Mate:184 (26.9875 mm): 47065T236_Silver Corner Bracket:4 ↔ 96282A101_High-Strength Steel Serrated Flange Locknut:5
- Mate:185 (26.9875 mm): 47065T236_Silver Corner Bracket:5 ↔ 96282A101_High-Strength Steel Serrated Flange Locknut:7
- Flush:186: 47065T236_Silver Corner Bracket:4 ↔ 47065T237_T-Slotted Framing:5
- Flush:187: 47065T237_T-Slotted Framing:5 ↔ 47065T237_T-Slotted Framing:4
- Mate:186 (12.7 mm): 47065T236_Silver Corner Bracket:6 ↔ 7779T391_Low-Carbon Steel U-Channel:1
- Flush:188: 47065T237_T-Slotted Framing:5 ↔ 47065T236_Silver Corner Bracket:6
- Flush:189: 47065T236_Silver Corner Bracket:4 ↔ 47065T236_Silver Corner Bracket:6
- Mate:187 (6.35 mm): QCI-34HC-3_v2:2 ↔ 47065T236_Silver Corner Bracket:7
- Mate:188 (41.275 mm): 47065T236_Silver Corner Bracket:7 ↔ ChassisInterface:2
- Flush:197 (6.35 mm): 47065T236_Silver Corner Bracket:3 ↔ ChassisInterface:2
- Mate:189: 47065T237_T-Slotted Framing:6 ↔ ChassisInterface:2
- Flush:198: 47065T236_Silver Corner Bracket:3 ↔ 47065T237_T-Slotted Framing:6
- Mate:190 (26.9875 mm): 47065T237_T-Slotted Framing:6 ↔ 96282A101_High-Strength Steel Serrated Flange Locknut:1
- Flush:202: 47065T237_T-Slotted Framing:5 ↔ 47065T237_T-Slotted Framing:8
- Flush:203: 47065T237_T-Slotted Framing:5 ↔ 47065T237_T-Slotted Framing:8
- Mate:191: 47065T237_T-Slotted Framing:8 ↔ TopPlate:2
- Mate:192: 47065T237_T-Slotted Framing:9 ↔ TopPlate:2
- Flush:204: 47065T237_T-Slotted Framing:8 ↔ 47065T237_T-Slotted Framing:9
- Flush:205: 47065T236_Silver Corner Bracket:7 ↔ 47065T237_T-Slotted Framing:9
- Mate:193 (28.575 mm): 47065T237_T-Slotted Framing:9 ↔ ChassisInterface:2
- Flush:206: 7779T391_Low-Carbon Steel U-Channel:1 ↔ OuterDriveRail:1
- Mate:194: 7779T391_Low-Carbon Steel U-Channel:1 ↔ OuterDriveRail:1
- Mate:195: 7779T391_Low-Carbon Steel U-Channel:1 ↔ InnerDriveRail:1
- Insert:51: 7779T391_Low-Carbon Steel U-Channel:1 ↔ InnerDriveRail:1
- Insert:52: 7779T391_Low-Carbon Steel U-Channel:1 ↔ InnerDriveRail:1
- Mate:196: 7779T391_Low-Carbon Steel U-Channel:1 ↔ OuterDriveRail:1
- Mate:197: TopPlate:2 ↔ ChassisInterface:2
- Flush:208: OuterDriveRail:1 ↔ TreadGuide:1
- Mate:198: OuterDriveRail:1 ↔ TreadGuide:1
- Mate:199: OuterDriveRail:1 ↔ TreadGuide:1
- Flush:209: 47065T237_T-Slotted Framing:5 ↔ 47065T237_T-Slotted Framing:6
- Flush:210: 47065T236_Silver Corner Bracket:7 ↔ 47065T237_T-Slotted Framing:6
- Mate:200: 47065T236_Silver Corner Bracket:8 ↔ InnerDriveRail:1
- Flush:211: 47065T236_Silver Corner Bracket:8 ↔ 47065T237_T-Slotted Framing:6
- Flush:212: 47065T236_Silver Corner Bracket:8 ↔ 47065T237_T-Slotted Framing:6
- Angle:41 (0 deg): ChassisInterface:2
- Tangent:1: V-Slot wheel:1
- Rotational:1 [RevoluteJoint]: 91263A553_Zinc-Plated Alloy Steel Hex Drive Flat Head Screw v1:2 ↔ TreadGuide:1
- Rotational:2 [RevoluteJoint]: 91263A553_Zinc-Plated Alloy Steel Hex Drive Flat Head Screw v1:3 ↔ TreadGuide:1
- Rotational:3 [RevoluteJoint]: 91263A553_Zinc-Plated Alloy Steel Hex Drive Flat Head Screw v1:4 ↔ TreadGuide:1
- Rotational:4 [RevoluteJoint]: 91263A553_Zinc-Plated Alloy Steel Hex Drive Flat Head Screw v1:5 ↔ TreadGuide:1
- Rotational:5 [RevoluteJoint]: 91263A553_Zinc-Plated Alloy Steel Hex Drive Flat Head Screw v1:1 ↔ TreadGuide:1
- Rotational:6 [RevoluteJoint]: 91263A553_Zinc-Plated Alloy Steel Hex Drive Flat Head Screw v1:6 ↔ TreadGuide:1
- Rotational:7 [RevoluteJoint]: 91263A553_Zinc-Plated Alloy Steel Hex Drive Flat Head Screw v1:7 ↔ TreadGuide:1
- Rotational:8 [RevoluteJoint]: 91263A553_Zinc-Plated Alloy Steel Hex Drive Flat Head Screw v1:8 ↔ TreadGuide:1
- Rotational:9 [RevoluteJoint]: 91263A553_Zinc-Plated Alloy Steel Hex Drive Flat Head Screw v1:9 ↔ TreadGuide:1
- Flush:213: driveshaftsupport_A:1 ↔ OuterDriveRail:1
- Flush:214: driveshaftsupport_A:1 ↔ OuterDriveRail:1
- Rotational:10 [RevoluteJoint]: 94328A911_Black Oxide Alloy Steel Low-Profile Shoulder Screw v2:2 ↔ OuterDriveRail:1
- Rotational:11 [RevoluteJoint]: 94328A911_Black Oxide Alloy Steel Low-Profile Shoulder Screw v2:1 ↔ OuterDriveRail:1
- Rotational:12 [RevoluteJoint]: 2868T203_High-Load Oil-Embedded 863 Sleeve Bearing:2 ↔ driveshaftsupport_A:1
- Rotational:13 [RevoluteJoint]: driveshaftsupport_A:2 ↔ OuterDriveRail:1
- Rotational:14 [RevoluteJoint]: 94328A911_Black Oxide Alloy Steel Low-Profile Shoulder Screw v2:4 ↔ OuterDriveRail:1
- Insert:53: 94328A911_Black Oxide Alloy Steel Low-Profile Shoulder Screw v2:3 ↔ OuterDriveRail:1
- Rotational:15 [RevoluteJoint]: 94328A911_Black Oxide Alloy Steel Low-Profile Shoulder Screw v2:3 ↔ OuterDriveRail:1
- Rotational:17 [RevoluteJoint] (90.805 mm): TankFlipper Flipped:1 ↔ rigid mount shoulder side:1
- Rotational:18 [RevoluteJoint] (-57.15 mm): TankFlipper:1 ↔ 6280K675_Roller Chain Sprocket:1
## Named parameters: d59_d55 = 0 mm, d60_d56 = 0 mm, d61_d57 = 0.6858 mm, d62_d58 = 0.6858 mm, d74_d69 = 3.175 mm, d335_d332 = 0 mm, d336_d333 = 0 mm, d337_d330 = 0 mm, d338_d331 = 0 mm, d360_d303 = 0 mm, d374_d369 = 0 mm, d375_d370 = 0 mm
